# Autodesk Inventor assembly: differential gearbox compact
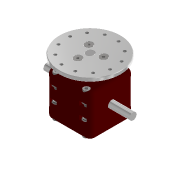
[picture p0: Inventor's stored thumbnail of the model, 180x180]
Saved by Autodesk Inventor 2020.3 (Build 243373000, 373)
## iProperties
Created: 2020-05-19
Part Number: differential gearbox compact
Document SubType Name: Assembly
Designer: stefa
Author: stefa
## Documents named in this file (17)
- C:\Users\Svend\OneDrive\Documents\GitHub\BeerMinder\3D-model\axis5_6\differential gearbox compact.iam
- C:\Users\Svend\OneDrive\Documents\GitHub\BeerMinder\3D-model\bearings\Ball Bearing 608ZZ.ipt
- C:\Users\Svend\OneDrive\Documents\GitHub\BeerMinder\3D-model\axis5_6\as bevelgear.ipt
- C:\Users\Svend\OneDrive\Documents\GitHub\BeerMinder\3D-model\axis5_6\tandwiel assemble.iam
- C:\Users\Svend\OneDrive\Documents\GitHub\BeerMinder\3D-model\axis5_6\gearbox v2.ipt
- C:\Users\Svend\OneDrive\Documents\GitHub\BeerMinder\3D-model\axis5_6\gearbox v2 mid part.ipt
- C:\Users\Svend\OneDrive\Documents\GitHub\BeerMinder\3D-model\axis5_6\as naar endeffector compact.ipt
- C:\Users\Svend\OneDrive\Documents\GitHub\BeerMinder\3D-model\axis5_6\endeffector mount as 8 compact.ipt
- C:\Users\Svend\OneDrive\Documents\GitHub\BeerMinder\3D-model\bearings\conische lager.ipt
- C:\Users\Svend\OneDrive\Documents\GitHub\BeerMinder\3D-model\axis5_6\conischLagerBlok.ipt
- C:\Users\Svend\OneDrive\Documents\GitHub\BeerMinder\3D-model\axis5_6\axis5_6 smaller v1\Design Accelerator\Bevel Gear11.ipt
- C:\Users\Svend\OneDrive\Documents\Inventor\Content Center Files\R2020\en-US\ISO 4035(2)\ISO 4035 - M4 - ISO.ipt
- C:\Users\Svend\OneDrive\Documents\Inventor\Content Center Files\R2020\en-US\ISO 4762(2)\ISO 4762 - M4 x 16ISO.ipt
- C:\Users\Svend\OneDrive\Documents\GitHub\BeerMinder\3D-model\axis4\asmountAs4.ipt
- C:\Users\Svend\OneDrive\Documents\GitHub\BeerMinder\3D-model\boutjesEnMoertjes\ISO 10642 - M4x12.ipt
- C:\Users\Svend\OneDrive\Documents\GitHub\BeerMinder\3D-model\ControlBox\swithces\mini microswitchDM1-02P.iam
- C:\Users\Svend\OneDrive\Documents\Inventor\Content Center Files\R2020\en-US\ISO 7380-1\ISO 7380-1 - M3 x 8.ipt
## Components (35 placed, 16 different names)
1. Ball Bearing 608ZZ:1 — Mate:30, Flush:14, Mate:37
2. Ball Bearing 608ZZ:2 — Mate:18, Mate:29, Flush:13
3. Ball Bearing 608ZZ:3 — Mate:23, Flush:10, Mate:24, Flush:20
4. as bevelgear:2 — Mate:18, Mate:33, Mate:40, Flush:19, Mate:51
5. as naar endeffector compact:1 — Mate:22, Flush:9, Angle:1, Mate:34, Flush:20, Mate:53, Tangent:1
6. endeffector mount as 8 compact:1 — Mate:22, Flush:9, Angle:1, Mate:44, Mate:45, Mate:46, Mate:47, Mate:48, Mate:49
7. tandwiel assemble:1 [sub-assembly] — Mate:24, Mate:34, Mate:38, Flush:18, Mate:42, Mate:50
8. gearbox v2:1 — Mate:23, Flush:10, Mate:26, Mate:27, Mate:28, Flush:11, Flush:12, Mate:31, Insert:12, Insert:13, Insert:14, Insert:15, Mate:52
9. gearbox v2 mid part:1 — Flush:11, Flush:12, Mate:29, Flush:13, Mate:30, Flush:14, Mate:31, Mate:33, Mate:35, Flush:15, Flush:16, Insert:1, Insert:2, Insert:3, Insert:4, Insert:5, Insert:6, Insert:7, Flush:21, Flush:22
10. conische lager:1 — Flush:17, Mate:43
11. conischLagerBlok:1 — Mate:35, Flush:15, Flush:16, Flush:17, Mate:43, Insert:8, Insert:9, Insert:10, Insert:11
12. as bevelgear:3 — Mate:37, Mate:38, Flush:18, Mate:50
13. Bevel Gear klein:1 — Mate:40, Flush:19, Mate:42, Mate:51
14. asmountAs4:1 — Mate:44, Mate:45, Mate:46
15. ISO 10642 M4x12:1 — Mate:47
16. ISO 10642 M4x12:2 — Mate:48
17. ISO 10642 M4x12:3 — Mate:49
18. mini microswitchDM1-02P:1 [sub-assembly] — Mate:52, Flush:21, Flush:22
19. ISO 7380-1 M3 x 8:1 — Mate:53, Tangent:1
20. ISO 4035 M4:3 — Insert:2
21. ISO 4035 M4:2 — Insert:1
22. ISO 4035 M4:4 — Insert:3
23. ISO 4035 M4:5 — Insert:4
24. ISO 4035 M4:8 — Insert:6
25. ISO 4035 M4:9 — Insert:7
26. ISO 4762 M4 x 16:1 — Insert:8
27. ISO 4762 M4 x 16:2 — Insert:9
28. ISO 4762 M4 x 16:3 — Insert:10
29. ISO 4762 M4 x 16:4 — Insert:11
30. ISO 4762 M4 x 16:5 — Insert:12
31. ISO 4762 M4 x 16:6 — Insert:13
32. ISO 4762 M4 x 16:7 — Insert:14
33. ISO 4762 M4 x 16:8 — Insert:15
34. ISO 4035 M4:6 — Insert:5
35. ISO 4035 M4:7
## Component patterns: (2 elements, first: ISO 4035 M4:6)
## Relationships (59: Mate 28, Insert 15, Flush 14, Angle 1, Tangent 1)
- Mate:18: Ball Bearing 608ZZ:2 ↔ as bevelgear:2
- Mate:22: as naar endeffector compact:1 ↔ endeffector mount as 8 compact:1
- Flush:9: as naar endeffector compact:1 ↔ endeffector mount as 8 compact:1
- Angle:1 (0 deg): as naar endeffector compact:1 ↔ endeffector mount as 8 compact:1
- Mate:23: Ball Bearing 608ZZ:3 ↔ gearbox v2:1
- Flush:10: Ball Bearing 608ZZ:3 ↔ gearbox v2:1
- Mate:24: Ball Bearing 608ZZ:3 ↔ tandwiel assemble:1
- Mate:26: gearbox v2:1
- Mate:27: gearbox v2:1
- Mate:28: gearbox v2:1
- Flush:11: gearbox v2:1 ↔ gearbox v2 mid part:1
- Flush:12: gearbox v2:1 ↔ gearbox v2 mid part:1
- Mate:29: Ball Bearing 608ZZ:2 ↔ gearbox v2 mid part:1
- Flush:13: Ball Bearing 608ZZ:2 ↔ gearbox v2 mid part:1
- Mate:30: Ball Bearing 608ZZ:1 ↔ gearbox v2 mid part:1
- Flush:14: Ball Bearing 608ZZ:1 ↔ gearbox v2 mid part:1
- Mate:31: gearbox v2:1 ↔ gearbox v2 mid part:1
- Mate:33: as bevelgear:2 ↔ gearbox v2 mid part:1
- Mate:34: as naar endeffector compact:1 ↔ tandwiel assemble:1
- Mate:35: gearbox v2 mid part:1 ↔ conischLagerBlok:1
- Flush:15: gearbox v2 mid part:1 ↔ conischLagerBlok:1
- Flush:16: gearbox v2 mid part:1 ↔ conischLagerBlok:1
- Flush:17: conische lager:1 ↔ conischLagerBlok:1
- Mate:37: Ball Bearing 608ZZ:1 ↔ as bevelgear:3
- Mate:38: tandwiel assemble:1 ↔ as bevelgear:3
- Flush:18: tandwiel assemble:1 ↔ as bevelgear:3
- Mate:40: as bevelgear:2 ↔ Bevel Gear klein:1
- Flush:19: as bevelgear:2 ↔ Bevel Gear klein:1
- Mate:42 (6.962 mm): tandwiel assemble:1 ↔ Bevel Gear klein:1
- Flush:20 (-10 mm): Ball Bearing 608ZZ:3 ↔ as naar endeffector compact:1
- Mate:43: conische lager:1 ↔ conischLagerBlok:1
- Insert:1: gearbox v2 mid part:1 ↔ ISO 4035 M4:2
- Insert:2: gearbox v2 mid part:1 ↔ ISO 4035 M4:3
- Insert:3: gearbox v2 mid part:1 ↔ ISO 4035 M4:4
- Insert:4: gearbox v2 mid part:1 ↔ ISO 4035 M4:5
- Insert:5: gearbox v2 mid part:1 ↔ ISO 4035 M4:6
- Insert:6: gearbox v2 mid part:1 ↔ ISO 4035 M4:8
- Insert:7: gearbox v2 mid part:1 ↔ ISO 4035 M4:9
- Insert:8: conischLagerBlok:1 ↔ ISO 4762 M4 x 16:1
- Insert:9: conischLagerBlok:1 ↔ ISO 4762 M4 x 16:2
- Insert:10: conischLagerBlok:1 ↔ ISO 4762 M4 x 16:3
- Insert:11: conischLagerBlok:1 ↔ ISO 4762 M4 x 16:4
- Insert:12: gearbox v2:1 ↔ ISO 4762 M4 x 16:5
- Insert:13: gearbox v2:1 ↔ ISO 4762 M4 x 16:6
- Insert:14: gearbox v2:1 ↔ ISO 4762 M4 x 16:7
- Insert:15: gearbox v2:1 ↔ ISO 4762 M4 x 16:8
- Mate:44: endeffector mount as 8 compact:1 ↔ asmountAs4:1
- Mate:45: endeffector mount as 8 compact:1 ↔ asmountAs4:1
- Mate:46: endeffector mount as 8 compact:1 ↔ asmountAs4:1
- Mate:47: endeffector mount as 8 compact:1 ↔ ISO 10642 M4x12:1
- Mate:48: endeffector mount as 8 compact:1 ↔ ISO 10642 M4x12:2
- Mate:49: endeffector mount as 8 compact:1 ↔ ISO 10642 M4x12:3
- Mate:50: tandwiel assemble:1 ↔ as bevelgear:3
- Mate:51: as bevelgear:2 ↔ Bevel Gear klein:1
- Mate:52: gearbox v2:1 ↔ mini microswitchDM1-02P:1
- Mate:53: as naar endeffector compact:1 ↔ ISO 7380-1 M3 x 8:1
- Tangent:1: as naar endeffector compact:1 ↔ ISO 7380-1 M3 x 8:1
- Flush:21 (10 mm): gearbox v2 mid part:1 ↔ mini microswitchDM1-02P:1
- Flush:22 (10 mm): gearbox v2 mid part:1 ↔ mini microswitchDM1-02P:1
